# Autodesk Inventor assembly: 26x30 VersaFrame
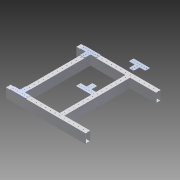
[picture p0: Inventor's stored thumbnail of the model, 180x180]
Saved by Autodesk Inventor 2015 (Build 190159000, 159)
## iProperties
Created: 2014-12-20
Part Number: 26x30 VersaFrame
Document SubType Name: Assembly
Designer: Nemo
Author: Nemo
## Documents named in this file (4)
- U:\26x30 Frame\26x30 VersaFrame 12-20-14.iam
- U:\26x30 Frame\VersaFrame End Rail 12-20-14.ipt
- U:\26x30 Frame\VersaFrame Side Rail 12-20-14.ipt
- U:\COTS Parts\VersaFrame\VersaFrame VersaChassis Gusset.ipt
## Components (8 placed, 5 different names)
1. VersaFrame End Rail: Front — Mate:1, Flush:1, Flush:2, Flush:3, Mate:6, Flush:14, Flush:18, Flush:19, Mate:10
2. VersaFrame End Rail: Back — Mate:1, Flush:2, Mate:4, Flush:10, Mate:9, Flush:22
3. VersaFrame Side Rail: Right — Flush:18, Mate:8, Flush:19, Flush:20, Flush:21
4. VersaFrame Side Rail 12-20-14:4 — Mate:9, Flush:22
5. VersaFrame VersaChassis Gusset:5
6. VersaFrame VersaChassis Gusset:6 — Mate:10
7. VersaFrame VersaChassis Gusset:2 — Mate:6, Flush:14, Flush:20
8. VersaFrame VersaChassis Gusset:4 — Mate:4, Flush:10, Flush:21
## Relationships (16: Flush 10, Mate 6)
- Mate:1: VersaFrame End Rail: Front ↔ VersaFrame End Rail: Back
- Flush:1 (52.3875 mm): VersaFrame End Rail: Front
- Flush:2: VersaFrame End Rail: Front ↔ VersaFrame End Rail: Back
- Flush:3: VersaFrame End Rail: Front
- Mate:4: VersaFrame End Rail: Back ↔ VersaFrame VersaChassis Gusset:4
- Flush:10: VersaFrame End Rail: Back ↔ VersaFrame VersaChassis Gusset:4
- Mate:6: VersaFrame End Rail: Front ↔ VersaFrame VersaChassis Gusset:2
- Flush:14: VersaFrame End Rail: Front ↔ VersaFrame VersaChassis Gusset:2
- Flush:18: VersaFrame End Rail: Front ↔ VersaFrame Side Rail: Right
- Mate:8: VersaFrame Side Rail: Right
- Flush:19 (50.8 mm): VersaFrame End Rail: Front ↔ VersaFrame Side Rail: Right
- Flush:20: VersaFrame Side Rail: Right ↔ VersaFrame VersaChassis Gusset:2
- Flush:21: VersaFrame Side Rail: Right ↔ VersaFrame VersaChassis Gusset:4
- Mate:9: VersaFrame End Rail: Back ↔ VersaFrame Side Rail 12-20-14:4
- Flush:22: VersaFrame End Rail: Back ↔ VersaFrame Side Rail 12-20-14:4
- Mate:10: VersaFrame End Rail: Front ↔ VersaFrame VersaChassis Gusset:6
## Named parameters: SideRailOffset = 50.8 mm, CenterDrop = 3.175 mm
